# Autodesk Inventor assembly: CIRCUIT_CASING
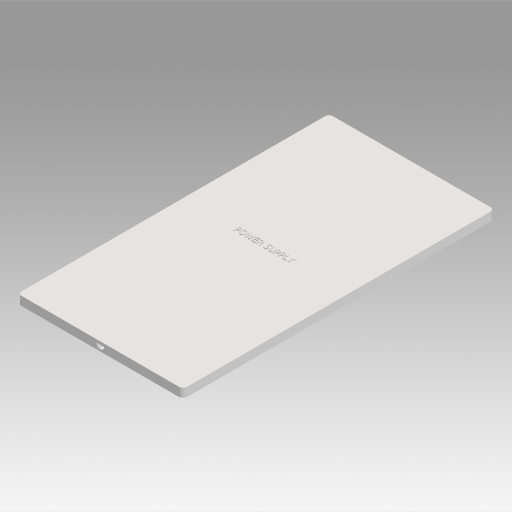
[picture p0: Inventor's stored thumbnail of the model, 512x512]
Saved by Autodesk Inventor 2023 (Build 270158000, 158)
## iProperties
Created: 2025-09-17
Part Number: CIRCUIT_CASING
Document SubType Name: Assembly
Designer: NELLY NDUNG'U
Author: NELLY NDUNG'U
## Documents named in this file (4)
- N:\NNW\PLC_PROJECTS\SPOTLIGHT PROJECT\CIRCUIT_CASING.iam
- N:\NNW\PLC_PROJECTS\SPOTLIGHT PROJECT\BOTTOM_COVER.ipt
- N:\NNW\PLC_PROJECTS\SPOTLIGHT PROJECT\PCB.ipt
- N:\NNW\PLC_PROJECTS\SPOTLIGHT PROJECT\TOP_COVER.ipt
## Components (3 placed, 3 different names)
1. BOTTOM_COVER:1 — Flush:1, Insert:1, Mate:1, Flush:2
2. PCB:1 — Insert:1
3. TOP_COVER:1 — Flush:1, Mate:1, Flush:2
## Relationships (4: Flush 2, Insert 1, Mate 1)
- Flush:1: BOTTOM_COVER:1 ↔ TOP_COVER:1
- Insert:1: BOTTOM_COVER:1 ↔ PCB:1
- Mate:1: BOTTOM_COVER:1 ↔ TOP_COVER:1
- Flush:2: BOTTOM_COVER:1 ↔ TOP_COVER:1
